# Autodesk Inventor assembly: Ensamblaje2
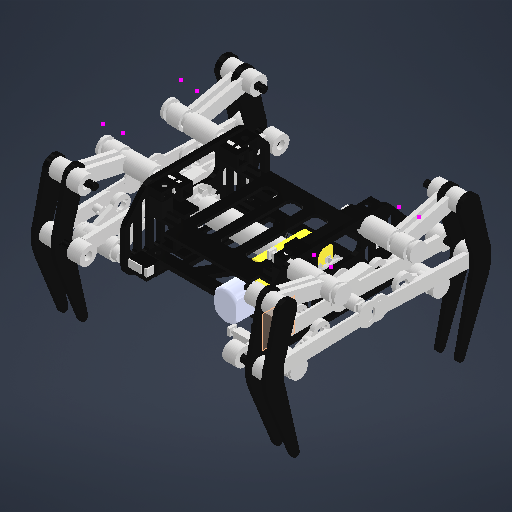
[picture p0: Inventor's stored thumbnail of the model, 512x512]
Saved by Autodesk Inventor 2026.1 (Build 301233020, 233B)
## iProperties
Created: 2025-11-20
Part Number: Ensamblaje2
Document SubType Name: Assembly
Designer: Asus
Author: Asus
## Documents named in this file (46)
- C:\UMNG\Semestre 6\Dinamica\Theo Jensen\Ensamblaje2.iam
- C:\UMNG\Semestre 6\Dinamica\Motor\Base_Superior_X1.ipt
- C:\UMNG\Semestre 6\Dinamica\Motor\Base_Izquierda_X1.ipt
- C:\UMNG\Semestre 6\Dinamica\Motor\Base_Derecha_X1.ipt
- C:\UMNG\Semestre 6\Dinamica\Motor\Base_Inferior_X1.ipt
- C:\UMNG\Semestre 6\Dinamica\Motor\Rodamiento_Motor_X2.ipt
- C:\UMNG\Semestre 6\Dinamica\Motor\Uniones_Planas_X2.ipt
- C:\UMNG\Semestre 6\Dinamica\Motor\Uniones_Planas_X2____2.ipt
- C:\UMNG\Semestre 6\Dinamica\Motor\Uniones_Planas_X2____3.ipt
- C:\UMNG\Semestre 6\Dinamica\Motor\Patas_X2.ipt
- C:\UMNG\Semestre 6\Dinamica\Motor\Motor\Motor.ipt
- C:\UMNG\Semestre 6\Dinamica\Motor\Rodamiento_Motor_Normal.ipt
- C:\UMNG\Semestre 6\Dinamica\Motor\Accesorios_X2__2.ipt
- C:\UMNG\Semestre 6\Dinamica\Motor\Palos_X4.ipt
- C:\UMNG\Semestre 6\Dinamica\Motor\Palos_X4_2.ipt
- C:\UMNG\Semestre 6\Dinamica\Motor\Uniones_Anchas_X2.ipt
- C:\UMNG\Semestre 6\Dinamica\Motor\Uniones_Anchas_X2_2.ipt
- C:\UMNG\Semestre 6\Dinamica\Motor\Uniones_Anchas_X2_3.ipt
- C:\UMNG\Semestre 6\Dinamica\Motor\Uniones_Planas_X2_MIR.ipt
- C:\UMNG\Semestre 6\Dinamica\Motor\Uniones_Planas_X2____2_MIR.ipt
- C:\UMNG\Semestre 6\Dinamica\Motor\Uniones_Planas_X2____3_MIR.ipt
- C:\UMNG\Semestre 6\Dinamica\Motor\Patas_X2_MIR.ipt
- C:\UMNG\Semestre 6\Dinamica\Motor\Accesorios_X2__2_MIR.ipt
- C:\UMNG\Semestre 6\Dinamica\Motor\Palos_X4_MIR.ipt
- C:\UMNG\Semestre 6\Dinamica\Motor\Palos_X4_2_MIR.ipt
- C:\UMNG\Semestre 6\Dinamica\Motor\Uniones_Anchas_X2_MIR.ipt
- C:\UMNG\Semestre 6\Dinamica\Motor\Uniones_Anchas_X2_2_MIR.ipt
- C:\UMNG\Semestre 6\Dinamica\Motor\Uniones_Anchas_X2_3_MIR.ipt
- C:\UMNG\Semestre 6\Dinamica\Motor\Uniones_Planas_X2_MIR1.ipt
- C:\UMNG\Semestre 6\Dinamica\Motor\Uniones_Planas_X2____2_MIR1.ipt
- C:\UMNG\Semestre 6\Dinamica\Motor\Uniones_Planas_X2____3_MIR1.ipt
- C:\UMNG\Semestre 6\Dinamica\Motor\Patas_X2_MIR1.ipt
- C:\UMNG\Semestre 6\Dinamica\Motor\Palos_X4_MIR1.ipt
- C:\UMNG\Semestre 6\Dinamica\Motor\Palos_X4_2_MIR1.ipt
- C:\UMNG\Semestre 6\Dinamica\Motor\Uniones_Anchas_X2_MIR1.ipt
- C:\UMNG\Semestre 6\Dinamica\Motor\Uniones_Anchas_X2_2_MIR1.ipt
- C:\UMNG\Semestre 6\Dinamica\Motor\Uniones_Anchas_X2_3_MIR1.ipt
- C:\UMNG\Semestre 6\Dinamica\Motor\Uniones_Planas_X2_MIR_MIR.ipt
- C:\UMNG\Semestre 6\Dinamica\Motor\Uniones_Planas_X2____2_MIR_MIR.ipt
- C:\UMNG\Semestre 6\Dinamica\Motor\Uniones_Planas_X2____3_MIR_MIR.ipt
- C:\UMNG\Semestre 6\Dinamica\Motor\Patas_X2_MIR_MIR.ipt
- C:\UMNG\Semestre 6\Dinamica\Motor\Palos_X4_MIR_MIR.ipt
- C:\UMNG\Semestre 6\Dinamica\Motor\Palos_X4_2_MIR_MIR.ipt
- C:\UMNG\Semestre 6\Dinamica\Motor\Uniones_Anchas_X2_MIR_MIR.ipt
- C:\UMNG\Semestre 6\Dinamica\Motor\Uniones_Anchas_X2_2_MIR_MIR.ipt
- C:\UMNG\Semestre 6\Dinamica\Motor\Uniones_Anchas_X2_3_MIR_MIR.ipt
## Components (49 placed, 45 different names)
1. Base_Superior_X1:1
2. Base_Izquierda_X1:1
3. Base_Derecha_X1:1
4. Base_Inferior_X1:1
5. Rodamiento_Motor_X2:1
6. Uniones_Planas_X2:1
7. Uniones_Planas_X2____2:1
8. Uniones_Planas_X2____3:1
9. Patas_X2:1
10. Motor:1
11. Rodamiento_Motor_Normal:1
12. Accesorios_X2__2:1 — Rígido:1
13. Patas_X2:2
14. Palos_X4:1
15. Palos_X4_2:1
16. Uniones_Anchas_X2:1
17. Uniones_Anchas_X2_2:1
18. Uniones_Anchas_X2_3:1 — Rígido:1
19. Uniones_Planas_X2_MIR:1
20. Uniones_Planas_X2____2_MIR:1
21. Uniones_Planas_X2____3_MIR:1
22. Patas_X2_MIR:1
23. Accesorios_X2__2_MIR:1 — Rígido:2
24. Patas_X2_MIR:2
25. Palos_X4_MIR:1
26. Palos_X4_2_MIR:1
27. Uniones_Anchas_X2_MIR:1
28. Uniones_Anchas_X2_2_MIR:1
29. Uniones_Anchas_X2_3_MIR:1 — Rígido:2
30. Uniones_Planas_X2_MIR1:1
31. Uniones_Planas_X2____2_MIR1:1
32. Uniones_Planas_X2____3_MIR1:1
33. Patas_X2_MIR1:1
34. Patas_X2_MIR1:2
35. Palos_X4_MIR1:1
36. Palos_X4_2_MIR1:1
37. Uniones_Anchas_X2_MIR1:1
38. Uniones_Anchas_X2_2_MIR1:1
39. Uniones_Anchas_X2_3_MIR1:1
40. Uniones_Planas_X2_MIR_MIR:1
41. Uniones_Planas_X2____2_MIR_MIR:1
42. Uniones_Planas_X2____3_MIR_MIR:1
43. Patas_X2_MIR_MIR:1
44. Patas_X2_MIR_MIR:2
45. Palos_X4_MIR_MIR:1
46. Palos_X4_2_MIR_MIR:1
47. Uniones_Anchas_X2_MIR_MIR:1
48. Uniones_Anchas_X2_2_MIR_MIR:1
49. Uniones_Anchas_X2_3_MIR_MIR:1
## Relationships (2: WeldJoint 2)
- Rígido:1 [WeldJoint]: Accesorios_X2__2:1 ↔ Uniones_Anchas_X2_3:1
- Rígido:2 [WeldJoint]: Accesorios_X2__2_MIR:1 ↔ Uniones_Anchas_X2_3_MIR:1
